# Autodesk Inventor assembly: bedMainAssembly
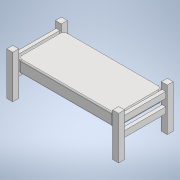
[picture p0: Inventor's stored thumbnail of the model, 180x180]
Saved by Autodesk Inventor 2022 (Build 260153000, 153)
## iProperties
Created: 2022-04-19
Part Number: bedMainAssembly
Document SubType Name: Assembly
Designer: compsci
Author: compsci
## Documents named in this file (3)
- C:\Users\compsci\Documents\VirtualPeddie\kayebed\bedMainAssembly.iam
- C:\Users\compsci\Documents\VirtualPeddie\kayebed\bed framehalf.iam
- C:\Users\compsci\Documents\VirtualPeddie\kayebed\mattress.ipt
## Components (3 placed, 2 different names)
1. bed framehalf:1 [sub-assembly] — Flush:1, Flush:2, Mate:2
2. bed framehalf:2 [sub-assembly] — Flush:1, Flush:2, Mate:1, Flush:3, Flush:4
3. mattress:1 — Mate:1, Mate:2, Flush:3, Flush:4
## Relationships (6: Flush 4, Mate 2)
- Flush:1: bed framehalf:1 ↔ bed framehalf:2
- Flush:2: bed framehalf:1 ↔ bed framehalf:2
- Mate:1: bed framehalf:2 ↔ mattress:1
- Mate:2: bed framehalf:1 ↔ mattress:1
- Flush:3 (76.2 mm): bed framehalf:2 ↔ mattress:1
- Flush:4: bed framehalf:2 ↔ mattress:1
